# Autodesk Inventor assembly: Green panel light assembly
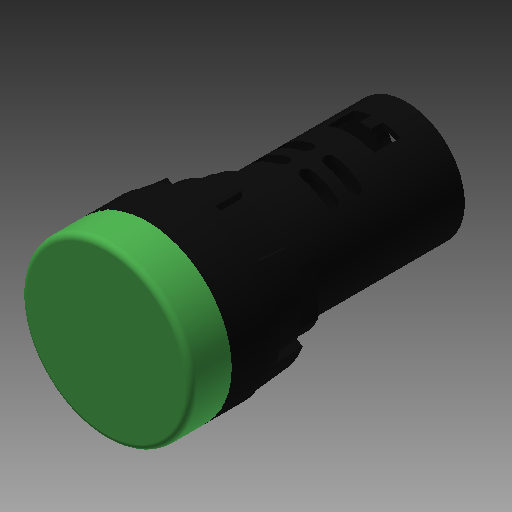
[picture p0: Inventor's stored thumbnail of the model, 512x512]
Saved by Autodesk Inventor 2017 (Build 210142000, 142)
## iProperties
Created: 2015-09-29
Part Number: Green panel light assembly
Document SubType Name: Assembly
Designer: USUARIO
Title: Green panel light assembly.STEP
Description: STEP AP214
Creation Date: 2015-05-16
Sending System: SolidWorks 2014
Preprocessor: SwSTEP 2.0
Author: USUARIO
## Documents named in this file (5)
- D:\UNAL\DISEÑO MECATRÓNICO\PARCIAL1\INTRODUCIBLES\BOMBILLOS\Green panel light assembly.iam
- D:\UNAL\DISEÑO MECATRÓNICO\PARCIAL1\INTRODUCIBLES\BOMBILLOS\light panel.ipt
- D:\UNAL\DISEÑO MECATRÓNICO\PARCIAL1\INTRODUCIBLES\BOMBILLOS\light green.ipt
- D:\UNAL\DISEÑO MECATRÓNICO\PARCIAL1\INTRODUCIBLES\BOMBILLOS\light nut.ipt
- D:\UNAL\DISEÑO MECATRÓNICO\PARCIAL1\INTRODUCIBLES\BOMBILLOS\light reflector.ipt
## Components (4 placed, 4 different names)
1. light panel_1 — Mate:1, Mate:2
2. light green_2
3. light nut_3 — Mate:1, Mate:2
4. light reflector_4
## Relationships (2: Mate 2)
- Mate:1: light panel_1 ↔ light nut_3
- Mate:2: light panel_1 ↔ light nut_3
